# Autodesk Inventor assembly: 80mm Gantry Set univseral
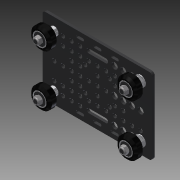
[picture p0: Inventor's stored thumbnail of the model, 180x180]
Saved by Autodesk Inventor 2014 SP1 (Build 180222100, 222)
## iProperties
Created: 2016-04-10
Part Number: 80mm Gantry Set univseral
Document SubType Name: Assembly
Designer: Ben
Author: Ben
## Documents named in this file (6)
- C:\Users\Ben\Documents\Autodesk\Projects\Me\3D printer\carriages\stp\Inventor\80mm Gantry Set univseral.iam
- C:\Users\Ben\Documents\Autodesk\Projects\Me\3D printer\carriages\stp\Inventor\80mm gantry plate.ipt
- C:\Users\Ben\Documents\Autodesk\Projects\Me\3D printer\carriages\stp\Inventor\V-Wheel Solid Wheel.iam
- C:\Users\Ben\Documents\Autodesk\Projects\Me\3D printer\carriages\stp\Inventor\V-Wheel Solid Wheel - spacer.iam
- C:\Users\Ben\Documents\Autodesk\Projects\Me\3D printer\carriages\stp\Inventor\M5x25 low profile screw.ipt
- C:\Users\Ben\Documents\Autodesk\Projects\Me\3D printer\carriages\stp\Inventor\M5 Nylock.ipt
## Components (13 placed, 5 different names)
1. 80mm gantry plate:1 — Mate:3, Mate:4, Mate:7, Mate:8, Mate:13, Mate:14, Mate:15, Mate:16, Flush:1, Mate:33, Mate:34, Mate:35, Mate:36, Flush:2, Flush:3
2. V-Wheel Solid Wheel:1 [sub-assembly] — Mate:8, Mate:23, Mate:32
3. V-Wheel Solid Wheel:2 [sub-assembly] — Mate:7, Mate:24, Mate:31
4. V-Wheel Solid Wheel - spacer:1 [sub-assembly] — Mate:3, Mate:21, Mate:26
5. V-Wheel Solid Wheel - spacer:2 [sub-assembly] — Mate:4, Mate:22, Mate:28
6. M5x25 low profile screw:1 — Mate:16, Mate:20, Mate:26, Mate:33
7. M5x25 low profile screw:2 — Mate:15, Mate:19, Mate:28, Mate:34
8. M5x25 low profile screw:3 — Mate:14, Mate:18, Mate:32, Mate:35
9. M5x25 low profile screw:4 — Mate:13, Mate:17, Mate:31, Mate:36
10. M5 Nylock:1 — Mate:20, Mate:21
11. M5 Nylock:2 — Mate:19, Mate:22
12. M5 Nylock:3 — Mate:18, Mate:23
13. M5 Nylock:4 — Mate:17, Mate:24
## Relationships (28: Mate 24, Flush 4)
- Mate:3: 80mm gantry plate:1 ↔ V-Wheel Solid Wheel - spacer:1
- Mate:4: 80mm gantry plate:1 ↔ V-Wheel Solid Wheel - spacer:2
- Mate:7: 80mm gantry plate:1 ↔ V-Wheel Solid Wheel:2
- Mate:8: 80mm gantry plate:1 ↔ V-Wheel Solid Wheel:1
- Mate:13: 80mm gantry plate:1 ↔ M5x25 low profile screw:4
- Mate:14: 80mm gantry plate:1 ↔ M5x25 low profile screw:3
- Mate:15: 80mm gantry plate:1 ↔ M5x25 low profile screw:2
- Mate:16: 80mm gantry plate:1 ↔ M5x25 low profile screw:1
- Mate:17: M5x25 low profile screw:4 ↔ M5 Nylock:4
- Mate:18: M5x25 low profile screw:3 ↔ M5 Nylock:3
- Mate:19: M5x25 low profile screw:2 ↔ M5 Nylock:2
- Mate:20: M5x25 low profile screw:1 ↔ M5 Nylock:1
- Mate:21: V-Wheel Solid Wheel - spacer:1 ↔ M5 Nylock:1
- Mate:22: V-Wheel Solid Wheel - spacer:2 ↔ M5 Nylock:2
- Mate:23: V-Wheel Solid Wheel:1 ↔ M5 Nylock:3
- Mate:24: V-Wheel Solid Wheel:2 ↔ M5 Nylock:4
- Mate:26: V-Wheel Solid Wheel - spacer:1 ↔ M5x25 low profile screw:1
- Mate:28: V-Wheel Solid Wheel - spacer:2 ↔ M5x25 low profile screw:2
- Mate:31: V-Wheel Solid Wheel:2 ↔ M5x25 low profile screw:4
- Mate:32: V-Wheel Solid Wheel:1 ↔ M5x25 low profile screw:3
- Flush:1 (11.885 mm): 80mm gantry plate:1
- Mate:33: 80mm gantry plate:1 ↔ M5x25 low profile screw:1
- Mate:34: 80mm gantry plate:1 ↔ M5x25 low profile screw:2
- Mate:35: 80mm gantry plate:1 ↔ M5x25 low profile screw:3
- Mate:36: 80mm gantry plate:1 ↔ M5x25 low profile screw:4
- Flush:2: 80mm gantry plate:1
- Flush:3: 80mm gantry plate:1
- Flush:4
